# Autodesk Inventor assembly: Montagem_Final
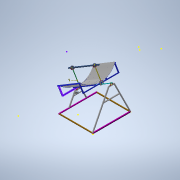
[picture p0: Inventor's stored thumbnail of the model, 180x180]
Saved by Autodesk Inventor 2022 (Build 260153000, 153)
## iProperties
Created: 2016-02-19
Part Number: Montagem_Final
Document SubType Name: Assembly
Designer: al131100X
Author: al131100X
## Documents named in this file (13)
- C:\Users\Alison\Documents\TCC\Peças e desenho no inventor - TCC\Peças\Montagem_Final.iam
- C:\Users\Alison\Documents\TCC\Desenhos e Montagem\desenhos e montagems inventor 15\METALON1.ipt
- C:\Users\Alison\Documents\TCC\Peças e desenho no inventor - TCC\Peças\CAVALETE_INFERIOR.ipt
- C:\Users\Alison\Documents\TCC\Peças e desenho no inventor - TCC\Peças\MONTAGEM_MANCAL.iam
- C:\Users\Alison\Documents\TCC\Peças e desenho no inventor - TCC\Peças\MONTAGEM_LAMINA_COM_SUPORTE.iam
- C:\Users\Alison\Documents\TCC\Desenhos e Montagem\desenhos e montagems inventor 15\metalon2.ipt
- C:\Users\Alison\Documents\TCC\Peças e desenho no inventor - TCC\Peças\CAVALETE_SUPERIOR.ipt
- C:\Users\Alison\Documents\TCC\Desenhos e Montagem\desenhos e montagems inventor 15\EIXO_30MM.ipt
- C:\Users\Alison\Documents\TCC\Peças e desenho no inventor - TCC\Peças\MONTAGEM_SUPORTE_ROLAMENTO.iam
- C:\Users\Alison\Documents\TCC\Peças e desenho no inventor - TCC\Peças\TUBO.ipt
- C:\Users\Alison\Documents\TCC\Desenhos e Montagem\Montagem motor correia e suporte.iam
- C:\Users\Alison\Documents\TCC\Peças e desenho no inventor - TCC\Peças\Montagem_Suporte_Rolamento_LDR.iam
- C:\Users\Alison\Documents\TCC\Peças e desenho no inventor - TCC\Peças\LDR.ipt
## Components (15 placed, 12 different names)
1. CAVALETE_INFERIOR:1 — Mate:11, Flush:11, Mate:12, Mate:21, Flush:16, Mate:25, Coincidente:46
2. MONTAGEM_MANCAL:2 [sub-assembly] — Mate:11, Flush:11, Mate:12, Mate:17, Mate:18
3. MONTAGEM_LAMINA_COM_SUPORTE:1 [sub-assembly] — Mate:17, Mate:18, Mate:19, Flush:22, Mate:30, Flush:23, Coincidente:47
4. MONTAGEM_MANCAL:3 [sub-assembly] — Mate:19, Mate:27, Flush:20, Mate:29, Coincidente:45
5. METALON1:1 — Mate:21, Mate:23, Flush:12, Flush:13, Mate:24, Flush:15, Flush:16, Mate:25, Flush:17, Flush:18
6. metalon2:1 — Mate:23, Flush:12, Flush:13, Flush:14
7. metalon2:2 — Flush:14, Mate:24, Flush:15, Flush:19, Mate:26
8. METALON1:2 — Flush:17, Flush:18, Flush:19, Mate:26, Flush:21, Mate:28, Coincidente:50
9. CAVALETE_SUPERIOR:1 — Mate:27, Flush:20, Flush:21, Mate:28, Coincidente:45, Coincidente:50
10. EIXO_30MM:1 — Mate:29, Coincidente:44
11. MONTAGEM_SUPORTE_ROLAMENTO:1 [sub-assembly] — Flush:22, Mate:30, Flush:23, Mate:43
12. TUBO:1 — Mate:43, Coincidente:48
13. Montagem motor correia e suporte:1 [sub-assembly] — Coincidente:44, Coincidente:46
14. Montagem_Suporte_Rolamento_LDR:1 [sub-assembly] — Coincidente:47, Coincidente:48, Inserir:1, Coincidente:49
15. LDR:1 — Inserir:1, Coincidente:49
## Relationships (36: Mate 22, Flush 13, Insert 1)
- Mate:11: CAVALETE_INFERIOR:1 ↔ MONTAGEM_MANCAL:2
- Flush:11: CAVALETE_INFERIOR:1 ↔ MONTAGEM_MANCAL:2
- Mate:12 (-85.9 mm): CAVALETE_INFERIOR:1 ↔ MONTAGEM_MANCAL:2
- Mate:17 (175 mm): MONTAGEM_MANCAL:2 ↔ MONTAGEM_LAMINA_COM_SUPORTE:1
- Mate:18: MONTAGEM_MANCAL:2 ↔ MONTAGEM_LAMINA_COM_SUPORTE:1
- Mate:19: MONTAGEM_LAMINA_COM_SUPORTE:1 ↔ MONTAGEM_MANCAL:3
- Mate:21: CAVALETE_INFERIOR:1 ↔ METALON1:1
- Mate:23: METALON1:1 ↔ metalon2:1
- Flush:12: METALON1:1 ↔ metalon2:1
- Flush:13: METALON1:1 ↔ metalon2:1
- Flush:14: metalon2:1 ↔ metalon2:2
- Mate:24: METALON1:1 ↔ metalon2:2
- Flush:15: METALON1:1 ↔ metalon2:2
- Flush:16: CAVALETE_INFERIOR:1 ↔ METALON1:1
- Mate:25: CAVALETE_INFERIOR:1 ↔ METALON1:1
- Flush:17: METALON1:1 ↔ METALON1:2
- Flush:18: METALON1:1 ↔ METALON1:2
- Flush:19: metalon2:2 ↔ METALON1:2
- Mate:26: metalon2:2 ↔ METALON1:2
- Mate:27: MONTAGEM_MANCAL:3 ↔ CAVALETE_SUPERIOR:1
- Flush:20: MONTAGEM_MANCAL:3 ↔ CAVALETE_SUPERIOR:1
- Flush:21: METALON1:2 ↔ CAVALETE_SUPERIOR:1
- Mate:28: METALON1:2 ↔ CAVALETE_SUPERIOR:1
- Mate:29: MONTAGEM_MANCAL:3 ↔ EIXO_30MM:1
- Flush:22 (65 mm): MONTAGEM_LAMINA_COM_SUPORTE:1 ↔ MONTAGEM_SUPORTE_ROLAMENTO:1
- Mate:30: MONTAGEM_LAMINA_COM_SUPORTE:1 ↔ MONTAGEM_SUPORTE_ROLAMENTO:1
- Flush:23 (822.25 mm): MONTAGEM_LAMINA_COM_SUPORTE:1 ↔ MONTAGEM_SUPORTE_ROLAMENTO:1
- Mate:43: MONTAGEM_SUPORTE_ROLAMENTO:1 ↔ TUBO:1
- Coincidente:44 [Mate]: EIXO_30MM:1 ↔ Montagem motor correia e suporte:1
- Coincidente:45 [Mate]: MONTAGEM_MANCAL:3 ↔ CAVALETE_SUPERIOR:1
- Coincidente:46 [Mate]: CAVALETE_INFERIOR:1 ↔ Montagem motor correia e suporte:1
- Coincidente:47 [Mate]: MONTAGEM_LAMINA_COM_SUPORTE:1 ↔ Montagem_Suporte_Rolamento_LDR:1
- Coincidente:48 [Mate]: TUBO:1 ↔ Montagem_Suporte_Rolamento_LDR:1
- Inserir:1: Montagem_Suporte_Rolamento_LDR:1 ↔ LDR:1
- Coincidente:49 [Mate]: Montagem_Suporte_Rolamento_LDR:1 ↔ LDR:1
- Coincidente:50 [Mate]: METALON1:2 ↔ CAVALETE_SUPERIOR:1
